# Autodesk Inventor assembly: 000.800 - Захват
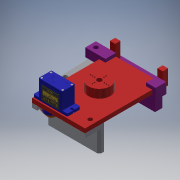
[picture p0: Inventor's stored thumbnail of the model, 180x180]
Saved by Autodesk Inventor 2019 (Build 230136000, 136)
## iProperties
Created: 2020-03-13
Part Number: 000.800 - Захват
Material: Типовые
Document SubType Name: Assembly
Designer: Петров Иван
Author: Петров Иван
## Documents named in this file (7)
- E:\IVAN\Ivan_desktop\Kvantorium\Competitions\INOP_2020\hardware\SCARA(Dynamixels)\000.600 - Захват.iam
- E:\IVAN\Ivan_desktop\Kvantorium\Competitions\INOP_2020\hardware\SCARA(Dynamixels)\000.601 - Опора.ipt
- E:\IVAN\Ivan_desktop\Kvantorium\Competitions\INOP_2020\hardware\SCARA(Dynamixels)\components\SG90 - Micro Servo 9g - Tower Pro.1.ipt
- E:\IVAN\Ivan_desktop\Kvantorium\Competitions\INOP_2020\hardware\SCARA(Dynamixels)\000.602 - Активный прижим.ipt
- E:\IVAN\Ivan_desktop\Kvantorium\Competitions\INOP_2020\hardware\SCARA(Dynamixels)\000.605 - Пассивный прижим.ipt
- E:\IVAN\Ivan_desktop\Kvantorium\Competitions\INOP_2020\hardware\SCARA(Dynamixels)\000.603 - Тяга.ipt
- E:\IVAN\Ivan_desktop\Kvantorium\Competitions\INOP_2020\hardware\SCARA(Dynamixels)\000.604 - Тяга.ipt
## Components (6 placed, 6 different names)
1. 000.601 - Опора:1 — Совмещение:1, Совмещение:2, Совмещение:3, Совмещение:4, Совмещение:5, Совмещение:6, Заподлицо:1, Совмещение:12
2. SG90 - Micro Servo 9g - Tower Pro.1:1 — Совмещение:1, Совмещение:2, Совмещение:3, Касательность:1, Совмещение:13, Совмещение:14
3. 000.602 - Активный прижим:1 — Совмещение:4, Совмещение:5, Совмещение:10, Совмещение:12
4. 000.605 - Пассивный прижим:1 — Совмещение:6, Заподлицо:1, Касательность:1
5. 000.603 - Тяга:1 — Совмещение:13, Совмещение:14, Совмещение:15, Совмещение:16
6. 000.604 - Тяга:1 — Совмещение:10, Совмещение:15, Совмещение:16
## Relationships (14: Mate 12, Flush 1, Tangent 1)
- Совмещение:1 [Mate]: 000.601 - Опора:1 ↔ SG90 - Micro Servo 9g - Tower Pro.1:1
- Совмещение:2 [Mate]: 000.601 - Опора:1 ↔ SG90 - Micro Servo 9g - Tower Pro.1:1
- Совмещение:3 [Mate]: 000.601 - Опора:1 ↔ SG90 - Micro Servo 9g - Tower Pro.1:1
- Совмещение:4 [Mate]: 000.601 - Опора:1 ↔ 000.602 - Активный прижим:1
- Совмещение:5 [Mate] (0.25 mm): 000.601 - Опора:1 ↔ 000.602 - Активный прижим:1
- Совмещение:6 [Mate]: 000.601 - Опора:1 ↔ 000.605 - Пассивный прижим:1
- Заподлицо:1 [Flush]: 000.601 - Опора:1 ↔ 000.605 - Пассивный прижим:1
- Касательность:1 [Tangent]: SG90 - Micro Servo 9g - Tower Pro.1:1 ↔ 000.605 - Пассивный прижим:1
- Совмещение:10 [Mate]: 000.602 - Активный прижим:1 ↔ 000.604 - Тяга:1
- Совмещение:12 [Mate]: 000.601 - Опора:1 ↔ 000.602 - Активный прижим:1
- Совмещение:13 [Mate]: SG90 - Micro Servo 9g - Tower Pro.1:1 ↔ 000.603 - Тяга:1
- Совмещение:14 [Mate]: SG90 - Micro Servo 9g - Tower Pro.1:1 ↔ 000.603 - Тяга:1
- Совмещение:15 [Mate]: 000.603 - Тяга:1 ↔ 000.604 - Тяга:1
- Совмещение:16 [Mate]: 000.603 - Тяга:1 ↔ 000.604 - Тяга:1
